# Autodesk Inventor assembly: _Design_SkimmerLid
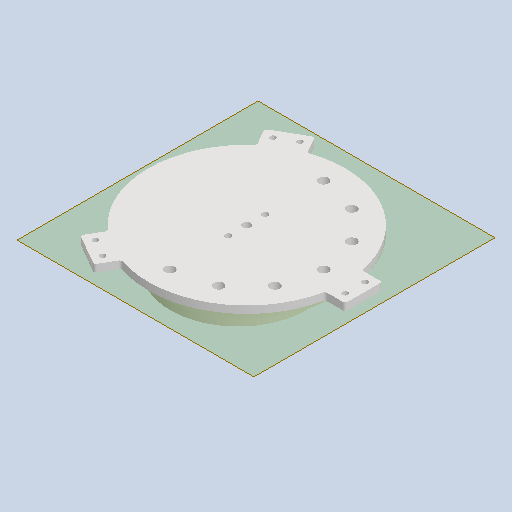
[picture p0: Inventor's stored thumbnail of the model, 512x512]
Saved by Autodesk Inventor 2023.2 (Build 272271030, 271C)
## iProperties
Created: 2023-02-16
Part Number: _Design_SkimmerLid
Document SubType Name: Assembly
Designer: atrus
Author: atrus
## Documents named in this file (3)
- C:\Users\atrus\Dropbox\elec\Mechanical\SkimmerSwabbie\_Design_SkimmerLid.iam
- C:\Users\atrus\Dropbox\elec\Mechanical\SkimmerSwabbie\SkimmerLid.ipt
- C:\Users\atrus\Dropbox\elec\Mechanical\SkimmerSwabbie\SkimmerLidInsert.ipt
## Components (2 placed, 2 different names)
1. SkimmerLid:1 — Insert:1
2. SkimmerLidInsert:1 — Insert:1
## Relationships (1: Insert 1)
- Insert:1: SkimmerLid:1 ↔ SkimmerLidInsert:1
